# Autodesk Inventor assembly: Assembly1
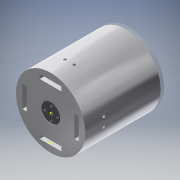
[picture p0: Inventor's stored thumbnail of the model, 180x180]
Saved by Autodesk Inventor 2016 (Build 200138000, 138)
## iProperties
Created: 2016-07-05
Part Number: Assembly1
Document SubType Name: Assembly
Designer: Andres
Author: Andres
## Documents named in this file (4)
- Z:\Documents\repositorios\BoreholeCamera\CAD_Probe\Enclosure\Assembly\Assembly1.iam
- Z:\Documents\repositorios\BoreholeCamera\CAD_Probe\Enclosure\Parts\Enclosure.ipt
- Z:\Documents\repositorios\BoreholeCamera\CAD_Probe\Enclosure\Parts\Cover.ipt
- Z:\Documents\repositorios\BoreholeCamera\CAD_Probe\Shaft Collar\SSCMN5b.ipt
## Components (3 placed, 3 different names)
1. Enclosure:1 — Rigid:1, Rigid:2
2. Cover:1 — Rigid:1
3. SSCMN5b:1 — Rigid:2
## Relationships (2: WeldJoint 2)
- Rigid:1 [WeldJoint]: Enclosure:1 ↔ Cover:1
- Rigid:2 [WeldJoint]: Enclosure:1 ↔ SSCMN5b:1
